# Autodesk Inventor assembly: full_layout_test
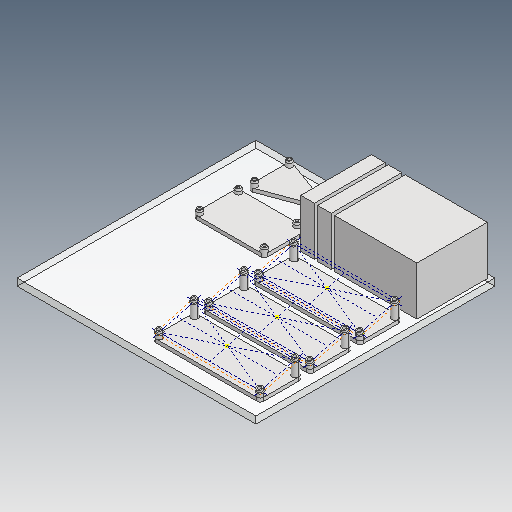
[picture p0: Inventor's stored thumbnail of the model, 512x512]
Saved by Autodesk Inventor 2025.4 (Build 294407020, 407B)
## iProperties
Created: 2026-09-08
Part Number: full_layout_test
Document SubType Name: Assembly
Designer: Aiden
Author: Aiden
## Documents named in this file (7)
- C:\Users\Aiden\Documents\GitHub\coldex-instrumentation\3d_models\mounting_hardware\dummy_parts\full_layout_test.iam
- C:\Users\Aiden\Documents\GitHub\coldex-instrumentation\3d_models\mounting_hardware\dummy_parts\acrylic_base.ipt
- C:\Users\Aiden\Documents\GitHub\coldex-instrumentation\3d_models\mounting_hardware\dummy_parts\din_pwr_supply.ipt
- C:\Users\Aiden\Documents\GitHub\coldex-instrumentation\3d_models\mounting_hardware\dummy_parts\din_voltage_regulator.ipt
- C:\Users\Aiden\Documents\GitHub\coldex-instrumentation\3d_models\mounting_hardware\arduino_mega_standoffs_plate.ipt
- C:\Users\Aiden\Documents\GitHub\coldex-instrumentation\3d_models\mounting_hardware\relay_module_standoffs_angled_plate.ipt
- C:\Users\Aiden\Documents\GitHub\coldex-instrumentation\3d_models\mounting_hardware\db-25_standoffs_plate.ipt
## Components (9 placed, 6 different names)
1. acrylic_base:1 — Mate:1, Mate:2, Mate:3, Mate:4, Mate:5, Mate:6
2. din_pwr_supply:1 — Mate:3
3. din_voltage_regulator:1 — Mate:2
4. din_voltage_regulator:2 — Mate:1
5. arduino_mega_standoffs_plate:1 — Mate:6
6. db-25_standoffs_plate:1 — Mate:5
7. relay_module_standoffs_angled_plate:1 — Mate:4
8. relay_module_standoffs_angled_plate:2
9. relay_module_standoffs_angled_plate:3
## Component patterns: (3 elements, first: relay_module_standoffs_angled_plate:1)
## Relationships (6: Mate 6)
- Mate:1: acrylic_base:1 ↔ din_voltage_regulator:2
- Mate:2: acrylic_base:1 ↔ din_voltage_regulator:1
- Mate:3: acrylic_base:1 ↔ din_pwr_supply:1
- Mate:4: acrylic_base:1 ↔ relay_module_standoffs_angled_plate:1
- Mate:5: acrylic_base:1 ↔ db-25_standoffs_plate:1
- Mate:6: acrylic_base:1 ↔ arduino_mega_standoffs_plate:1
